# Autodesk Inventor assembly: DeckelundGehäuse
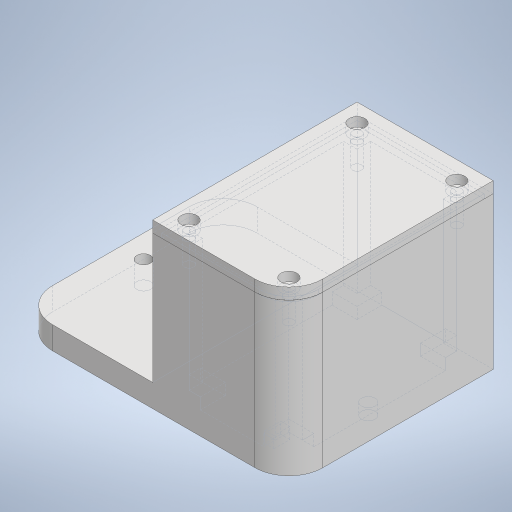
[picture p0: Inventor's stored thumbnail of the model, 512x512]
Saved by Autodesk Inventor 2024.2 (Build 282272000, 272)
## iProperties
Created: 2023-11-21
Part Number: DeckelundGehäuse
Document SubType Name: Assembly
Designer: Pieber
Author: Pieber
## Documents named in this file (3)
- C:\Users\Pieber\OneDrive - HTL Weiz\2023.24\Labor\Bergler\Zeitmessung\Halterung_Lichtschranke\DeckelundGehäuse.iam
- C:\Users\Pieber\OneDrive - HTL Weiz\2023.24\Labor\Bergler\Zeitmessung\Halterung_Lichtschranke\Gehäuse.ipt
- C:\Users\Pieber\OneDrive - HTL Weiz\2023.24\Labor\Bergler\Zeitmessung\Halterung_Lichtschranke\Deckel_Gehäuse.ipt
## Components (2 placed, 2 different names)
1. Gehäuse:1 — Starr:1
2. Deckel_Gehäuse:1 — Starr:1
## Relationships (1: WeldJoint 1)
- Starr:1 [WeldJoint]: Gehäuse:1 ↔ Deckel_Gehäuse:1
